# Autodesk Inventor assembly: hand3
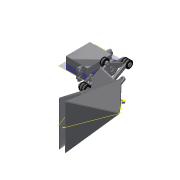
[picture p0: Inventor's stored thumbnail of the model, 180x180]
Saved by Autodesk Inventor 2019.4 (Build 234330000, 330)
## iProperties
Created: 2018-06-23
Part Number: hand3
Material: 一般
Document SubType Name: Assembly
Designer: AzLIer
Author: AzLIer
## Documents named in this file (13)
- E:\ロボ研\キャチロボ\キャチロボ2018\アーム\アーム01\hand03\hand3.iam
- E:\ロボ研\キャチロボ\キャチロボ2018\アーム\アーム01\hand01\Part4.ipt
- E:\ロボ研\キャチロボ\キャチロボ2018\アーム\アーム01\hand02\origami.iam
- E:\ロボ研\キャチロボ\キャチロボ2018\アーム\アーム01\hand03\Part100.ipt
- E:\ロボ研\キャチロボ\キャチロボ2018\アーム\アーム01\hand03\従動節固定.ipt
- E:\ロボ研\キャチロボ\キャチロボ2018\アーム\アーム01\hand03\link1.ipt
- E:\ロボ研\キャチロボ\キャチロボ2018\アーム\アーム01\hand03\φ6L5ジュラコン.ipt
- E:\ロボ研\キャチロボ\キャチロボ2018\アーム\アーム01\hand03\サーボホーンR.ipt
- E:\ロボ研\キャチロボ\キャチロボ2018\アーム\アーム01\hand03\p6t1ワッシャ.ipt
- E:\ロボ研\キャチロボ\キャチロボ2018\アーム\アーム01\hand03\link2.ipt
- E:\ロボ研\キャチロボ\キャチロボ2018\アーム\アーム01\hand03\hornLink.ipt
- E:\ロボ研\キャチロボ\キャチロボ2018\アーム\アーム01\hand03\handPlate.ipt
- E:\ロボ研\キャチロボ\キャチロボ2018\アーム\アーム01\hand03\handPlate2.ipt
## Components (28 placed, 12 different names)
1. Part4:1
2. Part100:1 — フラッシュ:1, メイト:23, メイト:24, メイト:37, 挿入:31, メイト:46
3. 従動節固定:1 — フラッシュ:1, メイト:23, メイト:24, メイト:35, 挿入:9
4. φ6L5ジュラコン:1 — メイト:35, 挿入:9, 挿入:10, 挿入:11
5. サーボホーンR:1 — メイト:37, 挿入:31, 挿入:32, メイト:39
6. origami:1 [sub-assembly] — メイト:41, メイト:43, メイト:44
7. link1:1 — 挿入:10, 挿入:12, 挿入:16, メイト:43, メイト:45, フラッシュ:2
8. p6t1ワッシャ:1 — 挿入:11
9. p6t1ワッシャ:2 — 挿入:12, 挿入:13, 挿入:14
10. link1:2 — 挿入:14, 挿入:15, 挿入:20, メイト:41, メイト:48, メイト:51
11. φ6L5ジュラコン:2 — 挿入:13, メイト:44, メイト:47
12. p6t1ワッシャ:3 — 挿入:15
13. link2:2 — 挿入:18, 挿入:19, メイト:38, 挿入:25
14. φ6L5ジュラコン:3 — 挿入:16, 挿入:17, 挿入:18
15. p6t1ワッシャ:4 — 挿入:17
16. p6t1ワッシャ:5 — 挿入:19
17. link2:1 — 挿入:21, 挿入:22, 挿入:23, メイト:38, 挿入:24, 挿入:26
18. φ6L5ジュラコン:4 — 挿入:20, 挿入:21
19. p6t1ワッシャ:6 — 挿入:22
20. p6t1ワッシャ:7 — 挿入:23
21. φ6L5ジュラコン:5 — 挿入:27, 挿入:28
22. p6t1ワッシャ:8 — 挿入:25
23. p6t1ワッシャ:9 — 挿入:24
24. p6t1ワッシャ:10 — 挿入:26, 挿入:27
25. φ6L5ジュラコン:6 — 挿入:28, メイト:40, メイト:46
26. hornLink:1 — 挿入:32, メイト:39, メイト:40
27. handPlate:1 — メイト:45, フラッシュ:2, メイト:47, メイト:50
28. handPlate2:1 — メイト:48, メイト:50, メイト:51
## Relationships (40: Insert 22, Mate 16, Flush 2)
- フラッシュ:1 [Flush] (5 mm): Part100:1 ↔ 従動節固定:1
- メイト:23 [Mate]: Part100:1 ↔ 従動節固定:1
- メイト:24 [Mate]: Part100:1 ↔ 従動節固定:1
- メイト:35 [Mate]: 従動節固定:1 ↔ φ6L5ジュラコン:1
- メイト:37 [Mate]: Part100:1 ↔ サーボホーンR:1
- 挿入:9 [Insert]: 従動節固定:1 ↔ φ6L5ジュラコン:1
- 挿入:10 [Insert] (-1 mm): φ6L5ジュラコン:1 ↔ link1:1
- 挿入:11 [Insert]: φ6L5ジュラコン:1 ↔ p6t1ワッシャ:1
- 挿入:12 [Insert]: link1:1 ↔ p6t1ワッシャ:2
- 挿入:13 [Insert]: p6t1ワッシャ:2 ↔ φ6L5ジュラコン:2
- 挿入:14 [Insert]: p6t1ワッシャ:2 ↔ link1:2
- 挿入:15 [Insert]: link1:2 ↔ p6t1ワッシャ:3
- 挿入:16 [Insert]: link1:1 ↔ φ6L5ジュラコン:3
- 挿入:17 [Insert]: φ6L5ジュラコン:3 ↔ p6t1ワッシャ:4
- 挿入:18 [Insert] (1 mm): link2:2 ↔ φ6L5ジュラコン:3
- 挿入:19 [Insert]: link2:2 ↔ p6t1ワッシャ:5
- 挿入:20 [Insert]: link1:2 ↔ φ6L5ジュラコン:4
- 挿入:21 [Insert] (1 mm): link2:1 ↔ φ6L5ジュラコン:4
- 挿入:22 [Insert]: link2:1 ↔ p6t1ワッシャ:6
- 挿入:23 [Insert]: link2:1 ↔ p6t1ワッシャ:7
- メイト:38 [Mate]: link2:2 ↔ link2:1
- 挿入:24 [Insert]: link2:1 ↔ p6t1ワッシャ:9
- 挿入:25 [Insert]: link2:2 ↔ p6t1ワッシャ:8
- 挿入:26 [Insert]: link2:1 ↔ p6t1ワッシャ:10
- 挿入:27 [Insert]: φ6L5ジュラコン:5 ↔ p6t1ワッシャ:10
- 挿入:28 [Insert]: φ6L5ジュラコン:5 ↔ φ6L5ジュラコン:6
- 挿入:31 [Insert]: Part100:1 ↔ サーボホーンR:1
- 挿入:32 [Insert]: サーボホーンR:1 ↔ hornLink:1
- メイト:39 [Mate]: サーボホーンR:1 ↔ hornLink:1
- メイト:40 [Mate]: φ6L5ジュラコン:6 ↔ hornLink:1
- メイト:41 [Mate]: origami:1 ↔ link1:2
- メイト:43 [Mate]: origami:1 ↔ link1:1
- メイト:44 [Mate]: origami:1 ↔ φ6L5ジュラコン:2
- メイト:45 [Mate]: link1:1 ↔ handPlate:1
- フラッシュ:2 [Flush]: link1:1 ↔ handPlate:1
- メイト:46 [Mate]: Part100:1 ↔ φ6L5ジュラコン:6
- メイト:47 [Mate]: φ6L5ジュラコン:2 ↔ handPlate:1
- メイト:48 [Mate]: link1:2 ↔ handPlate2:1
- メイト:50 [Mate]: handPlate:1 ↔ handPlate2:1
- メイト:51 [Mate]: link1:2 ↔ handPlate2:1
